# Autodesk Inventor assembly: PetriFilm
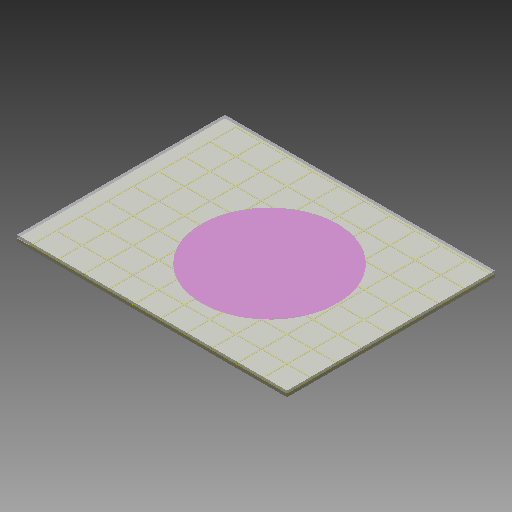
[picture p0: Inventor's stored thumbnail of the model, 512x512]
Saved by Autodesk Inventor 2019 (Build 230136000, 136)
## iProperties
Created: 2019-07-12
Part Number: PetriFilm
Document SubType Name: Assembly
Designer: Jorian Bruslind
Author: Jorian Bruslind
## Documents named in this file (3)
- C:\Users\Jorian Brusind\Documents\GitHub\ECE44x_Senior_Design\Design files\PetriFilm\PetriFilm.iam
- C:\Users\Jorian Brusind\Documents\GitHub\ECE44x_Senior_Design\Design files\PetriFilm\PetriFilm_WaxCover.ipt
- C:\Users\Jorian Brusind\Documents\GitHub\ECE44x_Senior_Design\Design files\PetriFilm\PetriFilm_Agar.ipt
## Components (2 placed, 2 different names)
1. PetriFilm_WaxCover:1 — Mate:1, Flush:1, Flush:2
2. PetriFilm_Agar:1 — Mate:1, Flush:1, Flush:2
## Relationships (3: Flush 2, Mate 1)
- Mate:1: PetriFilm_WaxCover:1 ↔ PetriFilm_Agar:1
- Flush:1: PetriFilm_WaxCover:1 ↔ PetriFilm_Agar:1
- Flush:2: PetriFilm_WaxCover:1 ↔ PetriFilm_Agar:1
